# Autodesk Inventor assembly: Octohedron
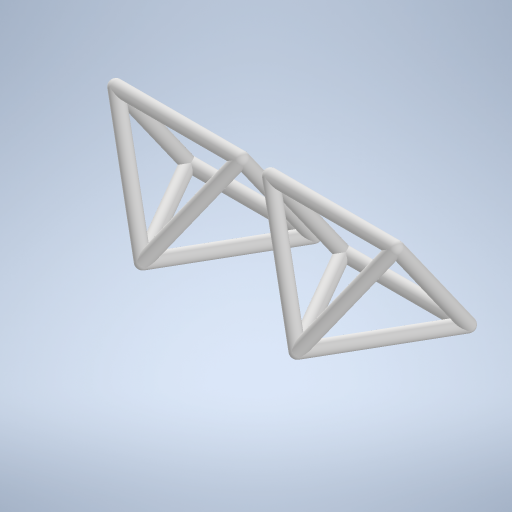
[picture p0: Inventor's stored thumbnail of the model, 512x512]
Saved by Autodesk Inventor 2023 (Build 270158000, 158)
## iProperties
Created: 2023-02-28
Part Number: Octohedron
Document SubType Name: Assembly
Designer: 100KStarsun
Author: 100KStarsun
## Documents named in this file (2)
- C:\Users\100ks\Documents\cwru\Think[Box]\Wire Octohedron\Octohedron.iam
- C:\Users\100ks\Documents\cwru\Think[Box]\Wire Octohedron\Pyramid.iam
## Components (2 placed, 1 different names)
1. Pyramid:1 [sub-assembly] — Flush:1, Flush:2
2. Pyramid:2 [sub-assembly] — Flush:1, Flush:2
## Relationships (2: Flush 2)
- Flush:1: Pyramid:1 ↔ Pyramid:2
- Flush:2: Pyramid:1 ↔ Pyramid:2
